# Autodesk Inventor assembly: Meraxes
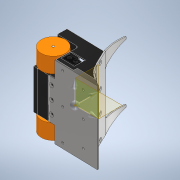
[picture p0: Inventor's stored thumbnail of the model, 180x180]
Saved by Autodesk Inventor 2021 (Build 250183000, 183)
## iProperties
Created: 2022-11-17
Part Number: Meraxes
Document SubType Name: Assembly
Designer: nicho
Mass: 388.653 g
Surface Area: 2241.89 cm^2
Volume: 523.873 cm^3
Density: 0.741883 g/cm^3
Author: nicho
## Documents named in this file (12)
- C:\Users\nicho\Documents\Work\RSM\Projetos Mecânicos\Meraxes\MK2\Meraxes.iam
- C:\Users\nicho\Documents\Work\RSM\Projetos Mecânicos\Meraxes\MK2\Peças Projetadas\Base Aço.ipt
- C:\Users\nicho\Documents\Work\RSM\Projetos Mecânicos\Meraxes\MK2\Peças Projetadas\Corpo.ipt
- C:\Users\nicho\Documents\Work\RSM\Projetos Mecânicos\Meraxes\MK2\Sistema Eletrônico\JS40F.ipt
- C:\Users\nicho\Documents\Work\RSM\Projetos Mecânicos\Meraxes\MK2\Sistema Eletrônico\Bateria 3S 650mAh.ipt
- C:\Users\nicho\Documents\Work\RSM\Projetos Mecânicos\Meraxes\MK2\Peças Projetadas\Apoio Motor.ipt
- C:\Users\nicho\Documents\Work\RSM\Projetos Mecânicos\Meraxes\MK2\Peças Compradas\Core-DC-motor-jsumo v1.ipt
- C:\Users\nicho\Documents\Work\RSM\Projetos Mecânicos\Meraxes\MK2\Peças Compradas\SLT20 v1.ipt
- C:\Users\nicho\Documents\Work\RSM\Projetos Mecânicos\Meraxes\MK2\Controle\Gabarito.ipt
- C:\Users\nicho\Documents\Work\RSM\Projetos Mecânicos\Meraxes\MK2\Peças Projetadas\Tampa Apoio Motor.ipt
- C:\Users\nicho\Documents\Work\RSM\Projetos Mecânicos\Meraxes\MK2\Controle\Alcance dos Sensores.ipt
- C:\Users\nicho\Documents\Work\RSM\Projetos Mecânicos\Meraxes\MK2\Peças Projetadas\Chapa Alumínio.ipt
## Components (21 placed, 11 different names)
1. Base Aço:1 — Coincidente:1, Coincidente:2, Coincidente:23, Coincidente:24, Coincidente:29
2. Corpo:1 — Coincidente:1, Coincidente:2, Coincidente:3, Coincidente:4, Coincidente:6, Coincidente:7, Coincidente:9, Coincidente:10, Coincidente:14, Coincidente:15, Coincidente:17, Coincidente:18, Coincidente:20, Coincidente:21, Coincidente:22, Coincidente:30, Coincidente:35, Coincidente:36, Coincidente:38, Coincidente:39, Coincidente:41, Coincidente:42, Coincidente:44, Coincidente:45, Coincidente:47, Coincidente:48, Coincidente:49, Coincidente:50, Coincidente:51, Coincidente:52, Coincidente:53, Coincidente:54, Coincidente:55, Alinhado:1, Alinhado:2
3. JS40F:1 — Coincidente:3, Coincidente:4, Coincidente:40, Coincidente:53
4. JS40F:2 — Coincidente:9, Coincidente:10, Coincidente:46, Coincidente:55
5. JS40F:3 — Coincidente:6, Coincidente:7, Coincidente:43, Coincidente:54
6. JS40F:4 — Coincidente:14, Coincidente:15, Coincidente:34, Alinhado:1
7. JS40F:5 — Coincidente:17, Coincidente:18, Coincidente:37, Alinhado:2
8. Bateria 3S 650mAh:1 — Coincidente:20, Coincidente:21, Coincidente:49
9. Apoio Motor:1 — Coincidente:22, Coincidente:23, Coincidente:24, Rígida:1, Rígida:2, Coincidente:31, Coincidente:32, Coincidente:33
10. Core-DC-motor-jsumo v1:1 — Rígida:1, Coincidente:25, Coincidente:26
11. Core-DC-motor-jsumo v1:2 — Rígida:2, Coincidente:27, Coincidente:28
12. SLT20 v1:1 — Coincidente:25, Coincidente:26, Tangente:1, Tangente:2
13. SLT20 v1:2 — Coincidente:27, Coincidente:28
14. Tampa Apoio Motor:1 — Coincidente:31, Coincidente:32, Coincidente:33
15. Chapa Alumínio:1 — Coincidente:50, Coincidente:51, Coincidente:52
16. Gabarito:1 — Tangente:1, Tangente:2, Coincidente:29, Coincidente:30
17. Alcance dos Sensores:1 — Coincidente:37, Coincidente:38, Coincidente:39
18. Alcance dos Sensores:2 — Coincidente:34, Coincidente:35, Coincidente:36
19. Alcance dos Sensores:3 — Coincidente:43, Coincidente:44, Coincidente:45
20. Alcance dos Sensores:4 — Coincidente:40, Coincidente:41, Coincidente:42
21. Alcance dos Sensores:5 — Coincidente:46, Coincidente:47, Coincidente:48
## Relationships (54: Mate 48, WeldJoint 2, Tangent 2, Flush 2)
- Coincidente:1 [Mate]: Base Aço:1 ↔ Corpo:1
- Coincidente:2 [Mate]: Base Aço:1 ↔ Corpo:1
- Coincidente:3 [Mate]: Corpo:1 ↔ JS40F:1
- Coincidente:4 [Mate] (0.65 mm): Corpo:1 ↔ JS40F:1
- Coincidente:6 [Mate]: Corpo:1 ↔ JS40F:3
- Coincidente:7 [Mate]: Corpo:1 ↔ JS40F:3
- Coincidente:9 [Mate]: Corpo:1 ↔ JS40F:2
- Coincidente:10 [Mate] (1.3 mm): Corpo:1 ↔ JS40F:2
- Coincidente:14 [Mate]: Corpo:1 ↔ JS40F:4
- Coincidente:15 [Mate]: Corpo:1 ↔ JS40F:4
- Coincidente:17 [Mate]: Corpo:1 ↔ JS40F:5
- Coincidente:18 [Mate]: Corpo:1 ↔ JS40F:5
- Coincidente:20 [Mate]: Corpo:1 ↔ Bateria 3S 650mAh:1
- Coincidente:21 [Mate]: Corpo:1 ↔ Bateria 3S 650mAh:1
- Coincidente:22 [Mate]: Corpo:1 ↔ Apoio Motor:1
- Coincidente:23 [Mate]: Base Aço:1 ↔ Apoio Motor:1
- Coincidente:24 [Mate]: Base Aço:1 ↔ Apoio Motor:1
- Rígida:1 [WeldJoint]: Apoio Motor:1 ↔ Core-DC-motor-jsumo v1:1
- Rígida:2 [WeldJoint]: Apoio Motor:1 ↔ Core-DC-motor-jsumo v1:2
- Coincidente:25 [Mate]: Core-DC-motor-jsumo v1:1 ↔ SLT20 v1:1
- Coincidente:26 [Mate]: Core-DC-motor-jsumo v1:1 ↔ SLT20 v1:1
- Coincidente:27 [Mate]: Core-DC-motor-jsumo v1:2 ↔ SLT20 v1:2
- Coincidente:28 [Mate]: Core-DC-motor-jsumo v1:2 ↔ SLT20 v1:2
- Tangente:1: SLT20 v1:1 ↔ Gabarito:1
- Tangente:2: SLT20 v1:1 ↔ Gabarito:1
- Coincidente:29 [Mate]: Base Aço:1 ↔ Gabarito:1
- Coincidente:30 [Mate]: Corpo:1 ↔ Gabarito:1
- Coincidente:31 [Mate]: Apoio Motor:1 ↔ Tampa Apoio Motor:1
- Coincidente:32 [Mate]: Apoio Motor:1 ↔ Tampa Apoio Motor:1
- Coincidente:33 [Mate]: Apoio Motor:1 ↔ Tampa Apoio Motor:1
- Coincidente:34 [Mate]: JS40F:4 ↔ Alcance dos Sensores:2
- Coincidente:35 [Mate]: Corpo:1 ↔ Alcance dos Sensores:2
- Coincidente:36 [Mate]: Corpo:1 ↔ Alcance dos Sensores:2
- Coincidente:37 [Mate]: JS40F:5 ↔ Alcance dos Sensores:1
- Coincidente:38 [Mate]: Corpo:1 ↔ Alcance dos Sensores:1
- Coincidente:39 [Mate]: Corpo:1 ↔ Alcance dos Sensores:1
- Coincidente:40 [Mate]: JS40F:1 ↔ Alcance dos Sensores:4
- Coincidente:41 [Mate]: Corpo:1 ↔ Alcance dos Sensores:4
- Coincidente:42 [Mate]: Corpo:1 ↔ Alcance dos Sensores:4
- Coincidente:43 [Mate]: JS40F:3 ↔ Alcance dos Sensores:3
- Coincidente:44 [Mate]: Corpo:1 ↔ Alcance dos Sensores:3
- Coincidente:45 [Mate]: Corpo:1 ↔ Alcance dos Sensores:3
- Coincidente:46 [Mate]: JS40F:2 ↔ Alcance dos Sensores:5
- Coincidente:47 [Mate]: Corpo:1 ↔ Alcance dos Sensores:5
- Coincidente:48 [Mate]: Corpo:1 ↔ Alcance dos Sensores:5
- Coincidente:49 [Mate] (5 mm): Corpo:1 ↔ Bateria 3S 650mAh:1
- Coincidente:50 [Mate]: Corpo:1 ↔ Chapa Alumínio:1
- Coincidente:51 [Mate]: Corpo:1 ↔ Chapa Alumínio:1
- Coincidente:52 [Mate]: Corpo:1 ↔ Chapa Alumínio:1
- Coincidente:53 [Mate]: Corpo:1 ↔ JS40F:1
- Coincidente:54 [Mate]: Corpo:1 ↔ JS40F:3
- Coincidente:55 [Mate]: Corpo:1 ↔ JS40F:2
- Alinhado:1 [Flush]: Corpo:1 ↔ JS40F:4
- Alinhado:2 [Flush]: Corpo:1 ↔ JS40F:5
